# Autodesk Inventor assembly: suspension_assy
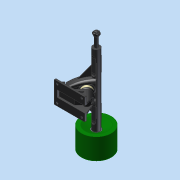
[picture p0: Inventor's stored thumbnail of the model, 180x180]
Saved by Autodesk Inventor 2015 SP1 (Build 190203100, 203)
## iProperties
Created: 2015-06-13
Part Number: suspension_assy
Document SubType Name: Assembly
Designer: YOUR_NAME_HERE
Author: nyikos.david
Title: C:\Users\nyikos.david\Documents\Rajzok\Grabcad\Longboard\suspension_assy.stp
Organization: TraceParts S.A.
Creation Date: 2015-06-01
Sending System: Autodesk Inventor 2015
Preprocessor: ST-DEVELOPER v15.6
Author: YOUR_NAME_HERE
## Documents named in this file (11)
- C:\Users\Rahul\Electric Skateboard\Electric Skateboard CAD\suspension_assy.iam
- C:\Users\Rahul\Electric Skateboard\Electric Skateboard CAD\Imported Components\suspension_assy\wheel_assy.iam
- C:\Users\Rahul\Electric Skateboard\Electric Skateboard CAD\Imported Components\suspension_assy\suspension.ipt
- C:\Users\Rahul\Electric Skateboard\Electric Skateboard CAD\Imported Components\suspension_assy\ISO 7719 - M8.ipt
- C:\Users\Rahul\Electric Skateboard\Electric Skateboard CAD\Imported Components\suspension_assy\suspension_part2.ipt
- C:\Users\Rahul\Electric Skateboard\Electric Skateboard CAD\Imported Components\suspension_assy\elasto_ring_1.ipt
- C:\Users\Rahul\Electric Skateboard\Electric Skateboard CAD\Imported Components\suspension_assy\elasto_ring_2.ipt
- C:\Users\Rahul\Electric Skateboard\Electric Skateboard CAD\Imported Components\suspension_assy\ring.ipt
- C:\Users\Rahul\Electric Skateboard\Electric Skateboard CAD\Imported Components\suspension_assy\ISO 4014 - M10 x 65DIN EN.ipt
- C:\Users\Rahul\Electric Skateboard\Electric Skateboard CAD\Imported Components\suspension_assy\ISO 4034 - M10DIN EN.ipt
- C:\Users\Rahul\Electric Skateboard\Electric Skateboard CAD\Imported Components\suspension_assy\ring_2.ipt
## Components (11 placed, 10 different names)
1. wheel_assy:1 [sub-assembly] — Mate:1, Mate:2
2. suspension:1 — Mate:1, Mate:2
3. ISO 7719 - M8:1
4. ISO 7719 - M8:2
5. suspension_part2:1
6. elasto_ring_1:1
7. elasto_ring_2:1
8. ring:1
9. ISO 4014 - M10 x 65DIN EN:1
10. ISO 4034 - M10DIN EN:1
11. ring_2:1
## Relationships (2: Mate 2)
- Mate:1: wheel_assy:1 ↔ suspension:1
- Mate:2: wheel_assy:1 ↔ suspension:1
